# Autodesk Inventor assembly: ruka
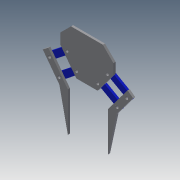
[picture p0: Inventor's stored thumbnail of the model, 180x180]
Saved by Autodesk Inventor 2013 (Build 170138000, 138)
## iProperties
Created: 2013-02-02
Part Number: ruka
Document SubType Name: Assembly
Designer: idle-rug
Author: idle-rug
## Documents named in this file (4)
- C:\Users\Petr\Documents\Inventor\robotic arm\ruka.iam
- C:\Users\Petr\Documents\Inventor\robotic arm\ruka_zak, deska.ipt
- C:\Users\Petr\Documents\Inventor\robotic arm\ruka_tahlo.ipt
- C:\Users\Petr\Documents\Inventor\robotic arm\packa1.ipt
## Components (7 placed, 3 different names)
1. ruka_zak, deska:1 — Mate:11, Mate:12, Mate:13, Mate:14, Mate:18, Mate:19, Mate:20, Mate:21
2. ruka_tahlo:6 — Mate:11, Mate:12, Mate:15, Mate:16
3. ruka_tahlo:7 — Mate:13, Mate:14, Mate:17
4. packa1:1 — Mate:15, Mate:16, Mate:17
5. packa1:2 — Mate:22, Mate:23, Mate:24
6. ruka_tahlo:8 — Mate:18, Mate:21, Mate:23
7. ruka_tahlo:9 — Mate:19, Mate:20, Mate:22, Mate:24
## Relationships (14: Mate 14)
- Mate:11: ruka_zak, deska:1 ↔ ruka_tahlo:6
- Mate:12: ruka_zak, deska:1 ↔ ruka_tahlo:6
- Mate:13: ruka_zak, deska:1 ↔ ruka_tahlo:7
- Mate:14: ruka_zak, deska:1 ↔ ruka_tahlo:7
- Mate:15: ruka_tahlo:6 ↔ packa1:1
- Mate:16: ruka_tahlo:6 ↔ packa1:1
- Mate:17: ruka_tahlo:7 ↔ packa1:1
- Mate:18: ruka_zak, deska:1 ↔ ruka_tahlo:8
- Mate:19: ruka_zak, deska:1 ↔ ruka_tahlo:9
- Mate:20: ruka_zak, deska:1 ↔ ruka_tahlo:9
- Mate:21: ruka_zak, deska:1 ↔ ruka_tahlo:8
- Mate:22: packa1:2 ↔ ruka_tahlo:9
- Mate:23: packa1:2 ↔ ruka_tahlo:8
- Mate:24: packa1:2 ↔ ruka_tahlo:9
